# Autodesk Inventor assembly: plugassmbly
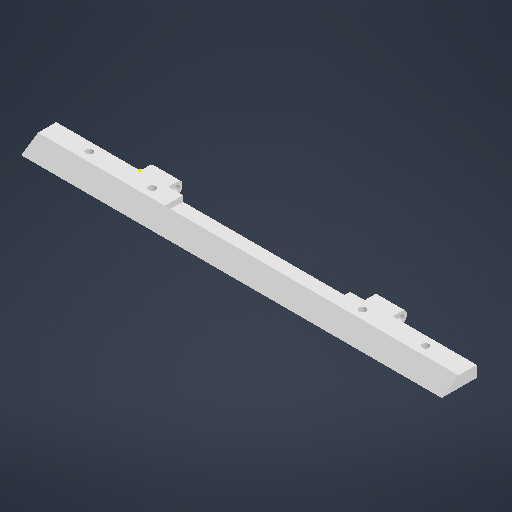
[picture p0: Inventor's stored thumbnail of the model, 512x512]
Saved by Autodesk Inventor 2026.2 (Build 302298010, 298A)
## iProperties
Created: 2026-05-09
Part Number: plugassmbly
Document SubType Name: Assembly
Designer: karol
Author: karol
## Documents named in this file (3)
- C:\Users\karol\OneDrive\Dokumenty\GitHub\bolt\bolt\cad\assembly\plugassmbly.iam
- C:\Users\karol\OneDrive\Dokumenty\GitHub\bolt\bolt\cad\ready parts\pługmoj.ipt
- C:\Users\karol\OneDrive\Dokumenty\GitHub\bolt\bolt\cad\ready parts\mocowanie do pługu.ipt
## Components (2 placed, 2 different names)
1. pługmoj:1 — Mate:1, Mate:2, Mate:3
2. mocowanie do pługu:1 — Mate:1, Mate:2, Mate:3
## Relationships (3: Mate 3)
- Mate:1: pługmoj:1 ↔ mocowanie do pługu:1
- Mate:2: pługmoj:1 ↔ mocowanie do pługu:1
- Mate:3: pługmoj:1 ↔ mocowanie do pługu:1
